(part 1 of 2)
# Autodesk Inventor assembly: 0008-10-01 Sckeleton
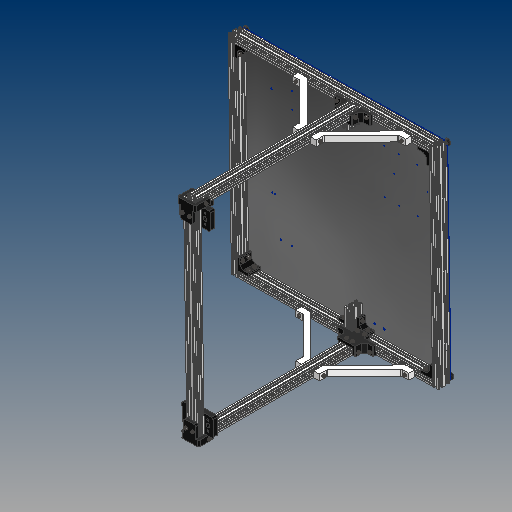
[picture p0: Inventor's stored thumbnail of the model, 512x512]
Saved by Autodesk Inventor 2020.2 (Build 242310000, 310)
## iProperties
Created: 2021-02-20
Part Number: 0008-10-01 Sckeleton
Document SubType Name: Assembly
Designer: Iulian Bors
Description: Scheleton
Author: Iulian Bors
Subject: 10-01
## Documents named in this file (20)
- Z:\I.A.B\Proiecte\0008 I.A.B 3D 2.1 Imprimanta aracet Metal\10 Mecanic\0008-10-01 Sckeleton.iam
- Z:\I.A.B\Proiecte\0008 I.A.B 3D 2.1 Imprimanta aracet Metal\10 Mecanic\0008-10-1018 V slot profiles.ipt
- Z:\I.A.B\Proiecte\0008 I.A.B 3D 2.1 Imprimanta aracet Metal\10 Mecanic\0008-10-1019 V slot profiles.ipt
- Z:\I.A.B\Proiecte\0008 I.A.B 3D 2.1 Imprimanta aracet Metal\10 Mecanic\0008-10-1020 V slot profiles.ipt
- Z:\I.A.B\Proiecte\0008 I.A.B 3D 2.1 Imprimanta aracet Metal\10 Mecanic\0008-10-1021  V slot profiles.ipt
- Z:\I.A.B\Proiecte\0008 I.A.B 3D 2.1 Imprimanta aracet Metal\10 Mecanic\0008-10-022 Tabla suport.ipt
- Z:\I.A.B\Proiecte\0008 I.A.B 3D 2.1 Imprimanta aracet Metal\10 Mecanic\0008-10-023 Suport L.ipt
- Z:\I.A.B\Proiecte\0008 I.A.B 3D 2.1 Imprimanta aracet Metal\10 Mecanic\0008-10-024 Ranforsare.ipt
- Z:\I.A.B\Proiecte\0008 I.A.B 3D 2.1 Imprimanta aracet Metal\10 Mecanic\0008-10-030 Suport L.ipt
- Z:\I.A.B\Proiecte\0008 I.A.B 3D 2.1 Imprimanta aracet Metal\10 Mecanic\0008-10-031 Suport L + placa.ipt
- Z:\I.A.B\Proiecte\0008 I.A.B 3D 2.1 Imprimanta aracet Metal\10 Mecanic\0008-10-032 Suport cadru si axa Z.ipt
- Z:\I.A.B\Proiecte\0008 I.A.B 3D 2.1 Imprimanta aracet Metal\10 Mecanic\0008-10-033.ipt
- Z:\I.A.B\Proiecte\0008 I.A.B 3D 2.1 Imprimanta aracet Metal\10 Mecanic\0008-10-035.ipt
- Z:\I.A.B\Proiecte\0008 I.A.B 3D 2.1 Imprimanta aracet Metal\10 Mecanic\0008-10-053 picior.ipt
- Z:\I.A.B\Proiecte\0008 I.A.B 3D 2.1 Imprimanta aracet Metal\10 Mecanic\0008-10-2010 M 5 Canal.ipt
- Z:\I.A.B\Proiecte\0008 I.A.B 3D 2.1 Imprimanta aracet Metal\10 Mecanic\0008-10-2011 DIN 7984 - M5 x 16.ipt
- Z:\I.A.B\Proiecte\0008 I.A.B 3D 2.1 Imprimanta aracet Metal\10 Mecanic\0008-10-2012 DIN 125 - A 5.3.ipt
- Z:\I.A.B\Proiecte\0008 I.A.B 3D 2.1 Imprimanta aracet Metal\10 Mecanic\0008-10-2013 DIN 7984 - M5 x 20.ipt
- Z:\I.A.B\Proiecte\0008 I.A.B 3D 2.1 Imprimanta aracet Metal\10 Mecanic\0008-10-2014 DIN 7984 - M5 x 25.ipt
- Z:\I.A.B\Proiecte\0008 I.A.B 3D 2.1 Imprimanta aracet Metal\10 Mecanic\0008-10-2015 DIN 7984 - M5 x 8.ipt
## Components (272 placed, 19 different names)
1. 0008-10-1018 V slot profiles.ipt:1 — Flush:78, Mate:85, Flush:79, Flush:80, Mate:86, Flush:81, Mate:109, Flush:101, Mate:112, Mate:114
2. 0008-10-1019 V slot profiles.ipt:2 — Flush:78, Mate:85, Flush:79, Mate:100, Flush:96, Mate:105, Flush:102, Mate:111, Flush:104, Mate:122, Mate:123, Flush:105, Mate:125, Flush:106, Mate:152, Mate:156, Mate:157
3. 0008-10-1019 V slot profiles.ipt:3 — Flush:80, Mate:86, Flush:81, Flush:82, Flush:85, Mate:90, Mate:99, Flush:95, Mate:106, Flush:100, Mate:116, Mate:119, Mate:127, Mate:132, Mate:143, Flush:114, Mate:146, Mate:149
4. 0008-10-1018 V slot profiles.ipt:4 — Flush:82, Flush:85, Mate:90, Flush:103, Mate:118, Mate:121
5. 0008-10-1018 V slot profiles.ipt:5 — Flush:97, Flush:98, Mate:110, Mate:161, Mate:165, Flush:116, Mate:170, Mate:177
6. 0008-10-1020 V slot profiles.ipt:6 — Flush:91, Mate:99, Flush:95, Flush:97, Flush:98, Mate:128, Flush:107, Mate:131, Flush:109, Mate:144, Mate:169, Flush:117, Flush:118, Mate:178
7. 0008-10-1020 V slot profiles.ipt:7 — Flush:91, Mate:100, Flush:96, Flush:103, Mate:110, Mate:124, Mate:126, Mate:158, Mate:159, Mate:162, Flush:115, Mate:166
8. 0008-10-1021  V slot profiles.ipt:8 — Mate:105, Mate:153, Mate:155, Flush:132
9. 0008-10-1021  V slot profiles.ipt:9 — Mate:106, Flush:100, Mate:147, Mate:150, Flush:132
10. 0008-10-022 Tabla suport.ipt:10 — Mate:109, Flush:101, Flush:102, Mate:115, Mate:117, Mate:120, Mate:145, Mate:148, Mate:151, Mate:154, Insert:21, Mate:179, Mate:180, Mate:181, Insert:242, Insert:265, Insert:266, Insert:267, Insert:268, Insert:269, Insert:270, Insert:271, Insert:272, Insert:273, Insert:274, Insert:275
11. 0008-10-023 Suport L.ipt:11 — Mate:111, Flush:104, Mate:112, Insert:24, Insert:33, Insert:34, Insert:35
12. 0008-10-023 Suport L.ipt:12 — Mate:120, Mate:121, Mate:122, Insert:66, Insert:67, Insert:68, Insert:69
13. 0008-10-023 Suport L.ipt:13 — Mate:117, Mate:118, Mate:119, Insert:54, Insert:55, Insert:56, Insert:57
14. 0008-10-023 Suport L.ipt:14 — Mate:114, Mate:115, Mate:116, Insert:36, Insert:43, Insert:44, Insert:45
15. 0008-10-024 Ranforsare.ipt:15 — Mate:123, Flush:105, Mate:124, Insert:235, Insert:236
16. 0008-10-024 Ranforsare.ipt:16 — Mate:127, Mate:128, Flush:107, Insert:224, Insert:227
17. 0008-10-024 Ranforsare.ipt:17 — Mate:125, Mate:126, Flush:106, Insert:237, Insert:239
18. 0008-10-024 Ranforsare.ipt:18 — Mate:131, Flush:109, Mate:132, Insert:230, Insert:231
19. 0008-10-031 Suport L + placa.ipt:19 — Mate:143, Mate:144, Flush:114, Insert:144, Insert:145, Insert:146, Insert:147, Insert:148, Insert:149, Insert:150, Insert:153
20. 0008-10-030 Suport L.ipt:20 — Mate:145, Mate:146, Mate:147, Insert:142, Insert:143
21. 0008-10-030 Suport L.ipt:21 — Mate:148, Mate:149, Mate:150, Insert:151, Insert:152
22. 0008-10-031 Suport L + placa.ipt:22 — Mate:157, Mate:158, Mate:159, Insert:96, Insert:97, Insert:98, Insert:99, Insert:100, Insert:101, Insert:102, Insert:103
23. 0008-10-030 Suport L.ipt:23 — Mate:151, Mate:152, Mate:153, Insert:94, Insert:95
24. 0008-10-030 Suport L.ipt:24 — Mate:154, Mate:155, Mate:156, Insert:104, Insert:105
25. 0008-10-032 Suport cadru si axa Z.ipt:25 — Mate:161, Mate:162, Flush:115, Insert:174, Insert:175, Insert:176, Insert:177
26. 0008-10-033.ipt:26 — Mate:165, Flush:116, Mate:166, Insert:197, Insert:198, Insert:199, Insert:200
27. 0008-10-035.ipt:27 — Mate:169, Flush:117, Mate:170, Insert:180, Mate:182, Insert:187, Insert:188
28. 0008-10-032 Suport cadru si axa Z.ipt:28 — Mate:177, Flush:118, Mate:178, Insert:162, Insert:163, Insert:164, Insert:165
29. 0008-10-053 picior.ipt:29 — Insert:21, Insert:115
30. 0008-10-053 picior.ipt:30 — Mate:181, Insert:116
31. 0008-10-053 picior.ipt:31 — Mate:179, Insert:117
32. 0008-10-053 picior.ipt:32 — Mate:180, Insert:114
33. 0008-10-2010 M 5 Canal.ipt:33 — Insert:22
34. 0008-10-2011 DIN 7984 - M5 x 16.ipt:34 — Insert:22, Insert:23
35. 0008-10-2012 DIN 125 - A 5.3.ipt:35 — Insert:23, Insert:24
36. 0008-10-2010 M 5 Canal.ipt:36
37. 0008-10-2011 DIN 7984 - M5 x 16.ipt:37
38. 0008-10-2012 DIN 125 - A 5.3.ipt:38 — Insert:33
39. 0008-10-2010 M 5 Canal.ipt:39
40. 0008-10-2011 DIN 7984 - M5 x 16.ipt:40
41. 0008-10-2012 DIN 125 - A 5.3.ipt:41 — Insert:34
42. 0008-10-2010 M 5 Canal.ipt:42
43. 0008-10-2011 DIN 7984 - M5 x 16.ipt:43
44. 0008-10-2012 DIN 125 - A 5.3.ipt:44 — Insert:35
45. 0008-10-2010 M 5 Canal.ipt:45
46. 0008-10-2011 DIN 7984 - M5 x 16.ipt:46
47. 0008-10-2012 DIN 125 - A 5.3.ipt:47 — Insert:36
48. 0008-10-2010 M 5 Canal.ipt:48
49. 0008-10-2011 DIN 7984 - M5 x 16.ipt:49
50. 0008-10-2012 DIN 125 - A 5.3.ipt:50 — Insert:44
51. 0008-10-2010 M 5 Canal.ipt:51
52. 0008-10-2011 DIN 7984 - M5 x 16.ipt:52
53. 0008-10-2012 DIN 125 - A 5.3.ipt:53 — Insert:45
54. 0008-10-2010 M 5 Canal.ipt:54
55. 0008-10-2011 DIN 7984 - M5 x 16.ipt:55
56. 0008-10-2012 DIN 125 - A 5.3.ipt:56 — Insert:43
57. 0008-10-2010 M 5 Canal.ipt:57
58. 0008-10-2011 DIN 7984 - M5 x 16.ipt:58
59. 0008-10-2012 DIN 125 - A 5.3.ipt:59 — Insert:57
60. 0008-10-2010 M 5 Canal.ipt:60
61. 0008-10-2011 DIN 7984 - M5 x 16.ipt:61
62. 0008-10-2012 DIN 125 - A 5.3.ipt:62 — Insert:56
63. 0008-10-2010 M 5 Canal.ipt:63
64. 0008-10-2011 DIN 7984 - M5 x 16.ipt:64
65. 0008-10-2012 DIN 125 - A 5.3.ipt:65 — Insert:55
66. 0008-10-2010 M 5 Canal.ipt:66
67. 0008-10-2011 DIN 7984 - M5 x 16.ipt:67
68. 0008-10-2012 DIN 125 - A 5.3.ipt:68 — Insert:54
69. 0008-10-2010 M 5 Canal.ipt:69
70. 0008-10-2011 DIN 7984 - M5 x 16.ipt:70
71. 0008-10-2012 DIN 125 - A 5.3.ipt:71 — Insert:66
72. 0008-10-2010 M 5 Canal.ipt:72
73. 0008-10-2011 DIN 7984 - M5 x 16.ipt:73
74. 0008-10-2012 DIN 125 - A 5.3.ipt:74 — Insert:67
75. 0008-10-2010 M 5 Canal.ipt:75
76. 0008-10-2011 DIN 7984 - M5 x 16.ipt:76
77. 0008-10-2012 DIN 125 - A 5.3.ipt:77 — Insert:68
78. 0008-10-2010 M 5 Canal.ipt:78
79. 0008-10-2011 DIN 7984 - M5 x 16.ipt:79
80. 0008-10-2012 DIN 125 - A 5.3.ipt:80 — Insert:69
81. 0008-10-2010 M 5 Canal.ipt:81
82. 0008-10-2011 DIN 7984 - M5 x 16.ipt:82
83. 0008-10-2012 DIN 125 - A 5.3.ipt:83 — Insert:94
84. 0008-10-2010 M 5 Canal.ipt:84
85. 0008-10-2011 DIN 7984 - M5 x 16.ipt:85
86. 0008-10-2012 DIN 125 - A 5.3.ipt:86 — Insert:96
87. 0008-10-2010 M 5 Canal.ipt:87
88. 0008-10-2011 DIN 7984 - M5 x 16.ipt:88
89. 0008-10-2012 DIN 125 - A 5.3.ipt:89 — Insert:95
90. 0008-10-2010 M 5 Canal.ipt:90
91. 0008-10-2011 DIN 7984 - M5 x 16.ipt:91
92. 0008-10-2012 DIN 125 - A 5.3.ipt:92 — Insert:97
93. 0008-10-2010 M 5 Canal.ipt:93
94. 0008-10-2011 DIN 7984 - M5 x 16.ipt:94
95. 0008-10-2012 DIN 125 - A 5.3.ipt:95 — Insert:98
96. 0008-10-2010 M 5 Canal.ipt:96
97. 0008-10-2011 DIN 7984 - M5 x 16.ipt:97
98. 0008-10-2012 DIN 125 - A 5.3.ipt:98 — Insert:102
99. 0008-10-2010 M 5 Canal.ipt:99
100. 0008-10-2011 DIN 7984 - M5 x 16.ipt:100
101. 0008-10-2012 DIN 125 - A 5.3.ipt:101 — Insert:100
102. 0008-10-2010 M 5 Canal.ipt:102
103. 0008-10-2011 DIN 7984 - M5 x 16.ipt:103
104. 0008-10-2012 DIN 125 - A 5.3.ipt:104 — Insert:101
105. 0008-10-2010 M 5 Canal.ipt:105
106. 0008-10-2011 DIN 7984 - M5 x 16.ipt:106
107. 0008-10-2012 DIN 125 - A 5.3.ipt:107 — Insert:105
108. 0008-10-2010 M 5 Canal.ipt:108
109. 0008-10-2011 DIN 7984 - M5 x 16.ipt:109
110. 0008-10-2012 DIN 125 - A 5.3.ipt:110 — Insert:104
111. 0008-10-2010 M 5 Canal.ipt:111
112. 0008-10-2011 DIN 7984 - M5 x 16.ipt:112
113. 0008-10-2012 DIN 125 - A 5.3.ipt:113 — Insert:103
114. 0008-10-2010 M 5 Canal.ipt:114
115. 0008-10-2011 DIN 7984 - M5 x 16.ipt:115
116. 0008-10-2012 DIN 125 - A 5.3.ipt:116 — Insert:99
117. 0008-10-2010 M 5 Canal.ipt:117
118. 0008-10-2011 DIN 7984 - M5 x 16.ipt:118
119. 0008-10-2012 DIN 125 - A 5.3.ipt:119 — Insert:114
120. 0008-10-2010 M 5 Canal.ipt:120
121. 0008-10-2011 DIN 7984 - M5 x 16.ipt:121
122. 0008-10-2012 DIN 125 - A 5.3.ipt:122 — Insert:115
123. 0008-10-2010 M 5 Canal.ipt:123
124. 0008-10-2011 DIN 7984 - M5 x 16.ipt:124
125. 0008-10-2012 DIN 125 - A 5.3.ipt:125 — Insert:116
126. 0008-10-2010 M 5 Canal.ipt:126
127. 0008-10-2011 DIN 7984 - M5 x 16.ipt:127
128. 0008-10-2012 DIN 125 - A 5.3.ipt:128 — Insert:117
129. 0008-10-2010 M 5 Canal.ipt:129
130. 0008-10-2011 DIN 7984 - M5 x 16.ipt:130
131. 0008-10-2012 DIN 125 - A 5.3.ipt:131 — Insert:145
132. 0008-10-2010 M 5 Canal.ipt:132
133. 0008-10-2011 DIN 7984 - M5 x 16.ipt:133
134. 0008-10-2012 DIN 125 - A 5.3.ipt:134 — Insert:144
135. 0008-10-2010 M 5 Canal.ipt:135
136. 0008-10-2011 DIN 7984 - M5 x 16.ipt:136
137. 0008-10-2012 DIN 125 - A 5.3.ipt:137 — Insert:143
138. 0008-10-2010 M 5 Canal.ipt:138
139. 0008-10-2011 DIN 7984 - M5 x 16.ipt:139
140. 0008-10-2012 DIN 125 - A 5.3.ipt:140 — Insert:146
141. 0008-10-2010 M 5 Canal.ipt:141
142. 0008-10-2011 DIN 7984 - M5 x 16.ipt:142
143. 0008-10-2012 DIN 125 - A 5.3.ipt:143 — Insert:150
144. 0008-10-2010 M 5 Canal.ipt:144
145. 0008-10-2011 DIN 7984 - M5 x 16.ipt:145
146. 0008-10-2012 DIN 125 - A 5.3.ipt:146 — Insert:147
147. 0008-10-2010 M 5 Canal.ipt:147
148. 0008-10-2011 DIN 7984 - M5 x 16.ipt:148
149. 0008-10-2012 DIN 125 - A 5.3.ipt:149 — Insert:153
150. 0008-10-2010 M 5 Canal.ipt:150
151. 0008-10-2011 DIN 7984 - M5 x 16.ipt:151
152. 0008-10-2012 DIN 125 - A 5.3.ipt:152 — Insert:152
153. 0008-10-2010 M 5 Canal.ipt:153
154. 0008-10-2011 DIN 7984 - M5 x 16.ipt:154
155. 0008-10-2012 DIN 125 - A 5.3.ipt:155 — Insert:151
156. 0008-10-2010 M 5 Canal.ipt:156
157. 0008-10-2011 DIN 7984 - M5 x 16.ipt:157
158. 0008-10-2012 DIN 125 - A 5.3.ipt:158 — Insert:149
159. 0008-10-2010 M 5 Canal.ipt:159
160. 0008-10-2011 DIN 7984 - M5 x 16.ipt:160
161. 0008-10-2012 DIN 125 - A 5.3.ipt:161 — Insert:148
162. 0008-10-2010 M 5 Canal.ipt:162
163. 0008-10-2011 DIN 7984 - M5 x 16.ipt:163
164. 0008-10-2012 DIN 125 - A 5.3.ipt:164 — Insert:142
165. 0008-10-2010 M 5 Canal.ipt:165
166. 0008-10-2011 DIN 7984 - M5 x 16.ipt:166
167. 0008-10-2012 DIN 125 - A 5.3.ipt:167 — Insert:162
168. 0008-10-2010 M 5 Canal.ipt:168
169. 0008-10-2011 DIN 7984 - M5 x 16.ipt:169
170. 0008-10-2012 DIN 125 - A 5.3.ipt:170 — Insert:163
171. 0008-10-2010 M 5 Canal.ipt:171
172. 0008-10-2011 DIN 7984 - M5 x 16.ipt:172
173. 0008-10-2012 DIN 125 - A 5.3.ipt:173 — Insert:165
174. 0008-10-2010 M 5 Canal.ipt:174
175. 0008-10-2011 DIN 7984 - M5 x 16.ipt:175
176. 0008-10-2012 DIN 125 - A 5.3.ipt:176 — Insert:164
177. 0008-10-2010 M 5 Canal.ipt:177
178. 0008-10-2011 DIN 7984 - M5 x 16.ipt:178
179. 0008-10-2012 DIN 125 - A 5.3.ipt:179 — Insert:174
180. 0008-10-2010 M 5 Canal.ipt:180
181. 0008-10-2011 DIN 7984 - M5 x 16.ipt:181
182. 0008-10-2012 DIN 125 - A 5.3.ipt:182 — Insert:176
183. 0008-10-2010 M 5 Canal.ipt:183
184. 0008-10-2011 DIN 7984 - M5 x 16.ipt:184
185. 0008-10-2012 DIN 125 - A 5.3.ipt:185 — Insert:175
186. 0008-10-2010 M 5 Canal.ipt:186
187. 0008-10-2011 DIN 7984 - M5 x 16.ipt:187
188. 0008-10-2012 DIN 125 - A 5.3.ipt:188 — Insert:177
189. 0008-10-2010 M 5 Canal.ipt:189 — Insert:178
190. 0008-10-2012 DIN 125 - A 5.3.ipt:190 — Insert:179, Insert:180
191. 0008-10-2013 DIN 7984 - M5 x 20.ipt:191 — Insert:178, Insert:179
192. 0008-10-2010 M 5 Canal.ipt:192
193. 0008-10-2012 DIN 125 - A 5.3.ipt:193 — Mate:182
194. 0008-10-2013 DIN 7984 - M5 x 20.ipt:194
195. 0008-10-2010 M 5 Canal.ipt:195
196. 0008-10-2012 DIN 125 - A 5.3.ipt:196 — Insert:188
197. 0008-10-2013 DIN 7984 - M5 x 20.ipt:197
198. 0008-10-2010 M 5 Canal.ipt:198
199. 0008-10-2012 DIN 125 - A 5.3.ipt:199 — Insert:187
200. 0008-10-2013 DIN 7984 - M5 x 20.ipt:200
201. 0008-10-2010 M 5 Canal.ipt:201
202. 0008-10-2012 DIN 125 - A 5.3.ipt:202 — Insert:198
203. 0008-10-2013 DIN 7984 - M5 x 20.ipt:203
204. 0008-10-2010 M 5 Canal.ipt:204
205. 0008-10-2012 DIN 125 - A 5.3.ipt:205 — Insert:200
206. 0008-10-2013 DIN 7984 - M5 x 20.ipt:206
207. 0008-10-2010 M 5 Canal.ipt:207
208. 0008-10-2012 DIN 125 - A 5.3.ipt:208 — Insert:199
209. 0008-10-2013 DIN 7984 - M5 x 20.ipt:209
210. 0008-10-2010 M 5 Canal.ipt:210
211. 0008-10-2012 DIN 125 - A 5.3.ipt:211 — Insert:197
212. 0008-10-2013 DIN 7984 - M5 x 20.ipt:212
213. 0008-10-2010 M 5 Canal.ipt:213
214. 0008-10-2010 M 5 Canal.ipt:214
215. 0008-10-2010 M 5 Canal.ipt:215
216. 0008-10-2010 M 5 Canal.ipt:216
217. 0008-10-2010 M 5 Canal.ipt:217
218. 0008-10-2012 DIN 125 - A 5.3.ipt:218 — Insert:224, Insert:225
219. 0008-10-2010 M 5 Canal.ipt:219
220. 0008-10-2010 M 5 Canal.ipt:220
221. 0008-10-2010 M 5 Canal.ipt:221
222. 0008-10-2014 DIN 7984 - M5 x 25.ipt:222 — Insert:225
223. 0008-10-2012 DIN 125 - A 5.3.ipt:223 — Insert:227
224. 0008-10-2014 DIN 7984 - M5 x 25.ipt:224
225. 0008-10-2012 DIN 125 - A 5.3.ipt:225 — Insert:231
226. 0008-10-2014 DIN 7984 - M5 x 25.ipt:226
227. 0008-10-2012 DIN 125 - A 5.3.ipt:227 — Insert:230
228. 0008-10-2014 DIN 7984 - M5 x 25.ipt:228
229. 0008-10-2012 DIN 125 - A 5.3.ipt:229 — Insert:237
230. 0008-10-2014 DIN 7984 - M5 x 25.ipt:230
231. 0008-10-2012 DIN 125 - A 5.3.ipt:231 — Insert:236
232. 0008-10-2014 DIN 7984 - M5 x 25.ipt:232
233. 0008-10-2012 DIN 125 - A 5.3.ipt:233 — Insert:235
234. 0008-10-2014 DIN 7984 - M5 x 25.ipt:234
235. 0008-10-2012 DIN 125 - A 5.3.ipt:235 — Insert:239
236. 0008-10-2014 DIN 7984 - M5 x 25.ipt:236
237. 0008-10-2010 M 5 Canal.ipt:237 — Insert:240
238. 0008-10-2012 DIN 125 - A 5.3.ipt:238 — Insert:241, Insert:242
239. 0008-10-2015 DIN 7984 - M5 x 8.ipt:239 — Insert:240, Insert:241
240. 0008-10-2010 M 5 Canal.ipt:240
241. 0008-10-2012 DIN 125 - A 5.3.ipt:241 — Insert:265
242. 0008-10-2015 DIN 7984 - M5 x 8.ipt:242
243. 0008-10-2010 M 5 Canal.ipt:243
244. 0008-10-2012 DIN 125 - A 5.3.ipt:244 — Insert:266
245. 0008-10-2015 DIN 7984 - M5 x 8.ipt:245
246. 0008-10-2010 M 5 Canal.ipt:246
247. 0008-10-2012 DIN 125 - A 5.3.ipt:247 — Insert:267
248. 0008-10-2015 DIN 7984 - M5 x 8.ipt:248
249. 0008-10-2010 M 5 Canal.ipt:249
250. 0008-10-2012 DIN 125 - A 5.3.ipt:250 — Insert:268
251. 0008-10-2015 DIN 7984 - M5 x 8.ipt:251
252. 0008-10-2010 M 5 Canal.ipt:252
253. 0008-10-2012 DIN 125 - A 5.3.ipt:253 — Insert:269
254. 0008-10-2015 DIN 7984 - M5 x 8.ipt:254
255. 0008-10-2010 M 5 Canal.ipt:255
256. 0008-10-2012 DIN 125 - A 5.3.ipt:256 — Insert:270
257. 0008-10-2015 DIN 7984 - M5 x 8.ipt:257
258. 0008-10-2010 M 5 Canal.ipt:258
259. 0008-10-2012 DIN 125 - A 5.3.ipt:259 — Insert:272
260. 0008-10-2015 DIN 7984 - M5 x 8.ipt:260
261. 0008-10-2010 M 5 Canal.ipt:261
262. 0008-10-2012 DIN 125 - A 5.3.ipt:262 — Insert:273
263. 0008-10-2015 DIN 7984 - M5 x 8.ipt:263
264. 0008-10-2010 M 5 Canal.ipt:264
265. 0008-10-2012 DIN 125 - A 5.3.ipt:265 — Insert:274
266. 0008-10-2015 DIN 7984 - M5 x 8.ipt:266
267. 0008-10-2010 M 5 Canal.ipt:267
268. 0008-10-2012 DIN 125 - A 5.3.ipt:268 — Insert:271
269. 0008-10-2015 DIN 7984 - M5 x 8.ipt:269
270. 0008-10-2010 M 5 Canal.ipt:270
271. 0008-10-2012 DIN 125 - A 5.3.ipt:271 — Insert:275
272. 0008-10-2015 DIN 7984 - M5 x 8.ipt:272
## Relationships (315: Insert 232, Mate 57, Flush 26)
- Flush:78: 0008-10-1018 V slot profiles.ipt:1 ↔ 0008-10-1019 V slot profiles.ipt:2
- Mate:85: 0008-10-1018 V slot profiles.ipt:1 ↔ 0008-10-1019 V slot profiles.ipt:2
- Flush:79: 0008-10-1018 V slot profiles.ipt:1 ↔ 0008-10-1019 V slot profiles.ipt:2
- Flush:80: 0008-10-1018 V slot profiles.ipt:1 ↔ 0008-10-1019 V slot profiles.ipt:3
- Mate:86: 0008-10-1018 V slot profiles.ipt:1 ↔ 0008-10-1019 V slot profiles.ipt:3
- Flush:81: 0008-10-1018 V slot profiles.ipt:1 ↔ 0008-10-1019 V slot profiles.ipt:3
- Flush:82: 0008-10-1019 V slot profiles.ipt:3 ↔ 0008-10-1018 V slot profiles.ipt:4
- Flush:85: 0008-10-1019 V slot profiles.ipt:3 ↔ 0008-10-1018 V slot profiles.ipt:4
- Mate:90: 0008-10-1019 V slot profiles.ipt:3 ↔ 0008-10-1018 V slot profiles.ipt:4
- Flush:91: 0008-10-1020 V slot profiles.ipt:6 ↔ 0008-10-1020 V slot profiles.ipt:7
- Mate:99: 0008-10-1019 V slot profiles.ipt:3 ↔ 0008-10-1020 V slot profiles.ipt:6
- Flush:95: 0008-10-1019 V slot profiles.ipt:3 ↔ 0008-10-1020 V slot profiles.ipt:6
- Mate:100: 0008-10-1019 V slot profiles.ipt:2 ↔ 0008-10-1020 V slot profiles.ipt:7
- Flush:96: 0008-10-1019 V slot profiles.ipt:2 ↔ 0008-10-1020 V slot profiles.ipt:7
- Flush:97: 0008-10-1018 V slot profiles.ipt:5 ↔ 0008-10-1020 V slot profiles.ipt:6
- Flush:98: 0008-10-1018 V slot profiles.ipt:5 ↔ 0008-10-1020 V slot profiles.ipt:6
- Mate:105: 0008-10-1019 V slot profiles.ipt:2 ↔ 0008-10-1021  V slot profiles.ipt:8
- Mate:106: 0008-10-1019 V slot profiles.ipt:3 ↔ 0008-10-1021  V slot profiles.ipt:9
- Flush:100: 0008-10-1019 V slot profiles.ipt:3 ↔ 0008-10-1021  V slot profiles.ipt:9
- Mate:109: 0008-10-1018 V slot profiles.ipt:1 ↔ 0008-10-022 Tabla suport.ipt:10
- Flush:101: 0008-10-1018 V slot profiles.ipt:1 ↔ 0008-10-022 Tabla suport.ipt:10
- Flush:102: 0008-10-1019 V slot profiles.ipt:2 ↔ 0008-10-022 Tabla suport.ipt:10
- Flush:103 (250.528 mm): 0008-10-1018 V slot profiles.ipt:4 ↔ 0008-10-1020 V slot profiles.ipt:7
- Mate:110: 0008-10-1018 V slot profiles.ipt:5 ↔ 0008-10-1020 V slot profiles.ipt:7
- Mate:111: 0008-10-1019 V slot profiles.ipt:2 ↔ 0008-10-023 Suport L.ipt:11
- Flush:104: 0008-10-1019 V slot profiles.ipt:2 ↔ 0008-10-023 Suport L.ipt:11
- Mate:112: 0008-10-1018 V slot profiles.ipt:1 ↔ 0008-10-023 Suport L.ipt:11
- Mate:114: 0008-10-1018 V slot profiles.ipt:1 ↔ 0008-10-023 Suport L.ipt:14
- Mate:115: 0008-10-022 Tabla suport.ipt:10 ↔ 0008-10-023 Suport L.ipt:14
- Mate:116: 0008-10-1019 V slot profiles.ipt:3 ↔ 0008-10-023 Suport L.ipt:14
- Mate:117: 0008-10-022 Tabla suport.ipt:10 ↔ 0008-10-023 Suport L.ipt:13
- Mate:118: 0008-10-1018 V slot profiles.ipt:4 ↔ 0008-10-023 Suport L.ipt:13
- Mate:119: 0008-10-1019 V slot profiles.ipt:3 ↔ 0008-10-023 Suport L.ipt:13
- Mate:120: 0008-10-022 Tabla suport.ipt:10 ↔ 0008-10-023 Suport L.ipt:12
- Mate:121: 0008-10-1018 V slot profiles.ipt:4 ↔ 0008-10-023 Suport L.ipt:12
- Mate:122: 0008-10-1019 V slot profiles.ipt:2 ↔ 0008-10-023 Suport L.ipt:12
- Mate:123: 0008-10-1019 V slot profiles.ipt:2 ↔ 0008-10-024 Ranforsare.ipt:15
- Flush:105: 0008-10-1019 V slot profiles.ipt:2 ↔ 0008-10-024 Ranforsare.ipt:15
- Mate:124: 0008-10-1020 V slot profiles.ipt:7 ↔ 0008-10-024 Ranforsare.ipt:15
- Mate:125: 0008-10-1019 V slot profiles.ipt:2 ↔ 0008-10-024 Ranforsare.ipt:17
- Mate:126: 0008-10-1020 V slot profiles.ipt:7 ↔ 0008-10-024 Ranforsare.ipt:17
- Flush:106: 0008-10-1019 V slot profiles.ipt:2 ↔ 0008-10-024 Ranforsare.ipt:17
- Mate:127: 0008-10-1019 V slot profiles.ipt:3 ↔ 0008-10-024 Ranforsare.ipt:16
- Mate:128: 0008-10-1020 V slot profiles.ipt:6 ↔ 0008-10-024 Ranforsare.ipt:16
- Flush:107: 0008-10-1020 V slot profiles.ipt:6 ↔ 0008-10-024 Ranforsare.ipt:16
- Mate:131: 0008-10-1020 V slot profiles.ipt:6 ↔ 0008-10-024 Ranforsare.ipt:18
- Flush:109: 0008-10-1020 V slot profiles.ipt:6 ↔ 0008-10-024 Ranforsare.ipt:18
- Mate:132: 0008-10-1019 V slot profiles.ipt:3 ↔ 0008-10-024 Ranforsare.ipt:18
- Mate:143: 0008-10-1019 V slot profiles.ipt:3 ↔ 0008-10-031 Suport L + placa.ipt:19
- Mate:144: 0008-10-1020 V slot profiles.ipt:6 ↔ 0008-10-031 Suport L + placa.ipt:19
- Flush:114: 0008-10-1019 V slot profiles.ipt:3 ↔ 0008-10-031 Suport L + placa.ipt:19
- Mate:145: 0008-10-022 Tabla suport.ipt:10 ↔ 0008-10-030 Suport L.ipt:20
- Mate:146: 0008-10-1019 V slot profiles.ipt:3 ↔ 0008-10-030 Suport L.ipt:20
- Mate:147: 0008-10-1021  V slot profiles.ipt:9 ↔ 0008-10-030 Suport L.ipt:20
- Mate:148: 0008-10-022 Tabla suport.ipt:10 ↔ 0008-10-030 Suport L.ipt:21
- Mate:149: 0008-10-1019 V slot profiles.ipt:3 ↔ 0008-10-030 Suport L.ipt:21
- Mate:150: 0008-10-1021  V slot profiles.ipt:9 ↔ 0008-10-030 Suport L.ipt:21
- Mate:151: 0008-10-022 Tabla suport.ipt:10 ↔ 0008-10-030 Suport L.ipt:23
- Mate:152: 0008-10-1019 V slot profiles.ipt:2 ↔ 0008-10-030 Suport L.ipt:23
- Mate:153: 0008-10-1021  V slot profiles.ipt:8 ↔ 0008-10-030 Suport L.ipt:23
- Mate:154: 0008-10-022 Tabla suport.ipt:10 ↔ 0008-10-030 Suport L.ipt:24
- Mate:155: 0008-10-1021  V slot profiles.ipt:8 ↔ 0008-10-030 Suport L.ipt:24
- Mate:156: 0008-10-1019 V slot profiles.ipt:2 ↔ 0008-10-030 Suport L.ipt:24
- Mate:157: 0008-10-1019 V slot profiles.ipt:2 ↔ 0008-10-031 Suport L + placa.ipt:22
- Mate:158: 0008-10-1020 V slot profiles.ipt:7 ↔ 0008-10-031 Suport L + placa.ipt:22
- Mate:159: 0008-10-1020 V slot profiles.ipt:7 ↔ 0008-10-031 Suport L + placa.ipt:22
- Mate:161: 0008-10-1018 V slot profiles.ipt:5 ↔ 0008-10-032 Suport cadru si axa Z.ipt:25
- Mate:162 (0.15 mm): 0008-10-1020 V slot profiles.ipt:7 ↔ 0008-10-032 Suport cadru si axa Z.ipt:25
- Flush:115: 0008-10-1020 V slot profiles.ipt:7 ↔ 0008-10-032 Suport cadru si axa Z.ipt:25
- Mate:165: 0008-10-1018 V slot profiles.ipt:5 ↔ 0008-10-033.ipt:26
- Flush:116: 0008-10-1018 V slot profiles.ipt:5 ↔ 0008-10-033.ipt:26
- Mate:166: 0008-10-1020 V slot profiles.ipt:7 ↔ 0008-10-033.ipt:26
- Mate:169: 0008-10-1020 V slot profiles.ipt:6 ↔ 0008-10-035.ipt:27
- Flush:117: 0008-10-1020 V slot profiles.ipt:6 ↔ 0008-10-035.ipt:27
- Mate:170: 0008-10-1018 V slot profiles.ipt:5 ↔ 0008-10-035.ipt:27
- Mate:177: 0008-10-1018 V slot profiles.ipt:5 ↔ 0008-10-032 Suport cadru si axa Z.ipt:28
- Flush:118: 0008-10-1020 V slot profiles.ipt:6 ↔ 0008-10-032 Suport cadru si axa Z.ipt:28
- Mate:178: 0008-10-1020 V slot profiles.ipt:6 ↔ 0008-10-032 Suport cadru si axa Z.ipt:28
- Flush:132: 0008-10-1021  V slot profiles.ipt:8 ↔ 0008-10-1021  V slot profiles.ipt:9
- Insert:21: 0008-10-022 Tabla suport.ipt:10 ↔ 0008-10-053 picior.ipt:29
- Mate:179: 0008-10-022 Tabla suport.ipt:10 ↔ 0008-10-053 picior.ipt:31
- Mate:180: 0008-10-022 Tabla suport.ipt:10 ↔ 0008-10-053 picior.ipt:32
- Mate:181: 0008-10-022 Tabla suport.ipt:10 ↔ 0008-10-053 picior.ipt:30
- Insert:22 (-5 mm): 0008-10-2010 M 5 Canal.ipt:33 ↔ 0008-10-2011 DIN 7984 - M5 x 16.ipt:34
- Insert:23: 0008-10-2011 DIN 7984 - M5 x 16.ipt:34 ↔ 0008-10-2012 DIN 125 - A 5.3.ipt:35
- Insert:24: 0008-10-023 Suport L.ipt:11 ↔ 0008-10-2012 DIN 125 - A 5.3.ipt:35
- [Insert] (-5 mm): 0008-10-2010 M 5 Canal.ipt:36 ↔ 0008-10-2011 DIN 7984 - M5 x 16.ipt:37
- [Insert]: 0008-10-2011 DIN 7984 - M5 x 16.ipt:37 ↔ 0008-10-2012 DIN 125 - A 5.3.ipt:38
- [Insert] (-5 mm): 0008-10-2010 M 5 Canal.ipt:39 ↔ 0008-10-2011 DIN 7984 - M5 x 16.ipt:40
- [Insert]: 0008-10-2011 DIN 7984 - M5 x 16.ipt:40 ↔ 0008-10-2012 DIN 125 - A 5.3.ipt:41
- [Insert] (-5 mm): 0008-10-2010 M 5 Canal.ipt:42 ↔ 0008-10-2011 DIN 7984 - M5 x 16.ipt:43
- [Insert]: 0008-10-2011 DIN 7984 - M5 x 16.ipt:43 ↔ 0008-10-2012 DIN 125 - A 5.3.ipt:44
- [Insert] (-5 mm): 0008-10-2010 M 5 Canal.ipt:45 ↔ 0008-10-2011 DIN 7984 - M5 x 16.ipt:46
- [Insert]: 0008-10-2011 DIN 7984 - M5 x 16.ipt:46 ↔ 0008-10-2012 DIN 125 - A 5.3.ipt:47
- Insert:33: 0008-10-023 Suport L.ipt:11 ↔ 0008-10-2012 DIN 125 - A 5.3.ipt:38
- Insert:34: 0008-10-023 Suport L.ipt:11 ↔ 0008-10-2012 DIN 125 - A 5.3.ipt:41
- Insert:35: 0008-10-023 Suport L.ipt:11 ↔ 0008-10-2012 DIN 125 - A 5.3.ipt:44
- Insert:36: 0008-10-023 Suport L.ipt:14 ↔ 0008-10-2012 DIN 125 - A 5.3.ipt:47
- [Insert] (-5 mm): 0008-10-2010 M 5 Canal.ipt:48 ↔ 0008-10-2011 DIN 7984 - M5 x 16.ipt:49
- [Insert]: 0008-10-2011 DIN 7984 - M5 x 16.ipt:49 ↔ 0008-10-2012 DIN 125 - A 5.3.ipt:50
- [Insert] (-5 mm): 0008-10-2010 M 5 Canal.ipt:51 ↔ 0008-10-2011 DIN 7984 - M5 x 16.ipt:52
- [Insert]: 0008-10-2011 DIN 7984 - M5 x 16.ipt:52 ↔ 0008-10-2012 DIN 125 - A 5.3.ipt:53
- [Insert] (-5 mm): 0008-10-2010 M 5 Canal.ipt:54 ↔ 0008-10-2011 DIN 7984 - M5 x 16.ipt:55
- [Insert]: 0008-10-2011 DIN 7984 - M5 x 16.ipt:55 ↔ 0008-10-2012 DIN 125 - A 5.3.ipt:56
- Insert:43: 0008-10-023 Suport L.ipt:14 ↔ 0008-10-2012 DIN 125 - A 5.3.ipt:56
- Insert:44: 0008-10-023 Suport L.ipt:14 ↔ 0008-10-2012 DIN 125 - A 5.3.ipt:50
- Insert:45: 0008-10-023 Suport L.ipt:14 ↔ 0008-10-2012 DIN 125 - A 5.3.ipt:53
- [Insert] (-5 mm): 0008-10-2010 M 5 Canal.ipt:57 ↔ 0008-10-2011 DIN 7984 - M5 x 16.ipt:58
- [Insert]: 0008-10-2011 DIN 7984 - M5 x 16.ipt:58 ↔ 0008-10-2012 DIN 125 - A 5.3.ipt:59
- [Insert] (-5 mm): 0008-10-2010 M 5 Canal.ipt:60 ↔ 0008-10-2011 DIN 7984 - M5 x 16.ipt:61
- [Insert]: 0008-10-2011 DIN 7984 - M5 x 16.ipt:61 ↔ 0008-10-2012 DIN 125 - A 5.3.ipt:62
- [Insert] (-5 mm): 0008-10-2010 M 5 Canal.ipt:63 ↔ 0008-10-2011 DIN 7984 - M5 x 16.ipt:64
- [Insert]: 0008-10-2011 DIN 7984 - M5 x 16.ipt:64 ↔ 0008-10-2012 DIN 125 - A 5.3.ipt:65
- [Insert] (-5 mm): 0008-10-2010 M 5 Canal.ipt:66 ↔ 0008-10-2011 DIN 7984 - M5 x 16.ipt:67
- [Insert]: 0008-10-2011 DIN 7984 - M5 x 16.ipt:67 ↔ 0008-10-2012 DIN 125 - A 5.3.ipt:68
- Insert:54: 0008-10-023 Suport L.ipt:13 ↔ 0008-10-2012 DIN 125 - A 5.3.ipt:68
- Insert:55: 0008-10-023 Suport L.ipt:13 ↔ 0008-10-2012 DIN 125 - A 5.3.ipt:65
- Insert:56: 0008-10-023 Suport L.ipt:13 ↔ 0008-10-2012 DIN 125 - A 5.3.ipt:62
- Insert:57: 0008-10-023 Suport L.ipt:13 ↔ 0008-10-2012 DIN 125 - A 5.3.ipt:59
- [Insert] (-5 mm): 0008-10-2010 M 5 Canal.ipt:69 ↔ 0008-10-2011 DIN 7984 - M5 x 16.ipt:70
- [Insert]: 0008-10-2011 DIN 7984 - M5 x 16.ipt:70 ↔ 0008-10-2012 DIN 125 - A 5.3.ipt:71
- [Insert] (-5 mm): 0008-10-2010 M 5 Canal.ipt:72 ↔ 0008-10-2011 DIN 7984 - M5 x 16.ipt:73
- [Insert]: 0008-10-2011 DIN 7984 - M5 x 16.ipt:73 ↔ 0008-10-2012 DIN 125 - A 5.3.ipt:74
- [Insert] (-5 mm): 0008-10-2010 M 5 Canal.ipt:75 ↔ 0008-10-2011 DIN 7984 - M5 x 16.ipt:76
- [Insert]: 0008-10-2011 DIN 7984 - M5 x 16.ipt:76 ↔ 0008-10-2012 DIN 125 - A 5.3.ipt:77
- [Insert] (-5 mm): 0008-10-2010 M 5 Canal.ipt:78 ↔ 0008-10-2011 DIN 7984 - M5 x 16.ipt:79
- [Insert]: 0008-10-2011 DIN 7984 - M5 x 16.ipt:79 ↔ 0008-10-2012 DIN 125 - A 5.3.ipt:80
- Insert:66: 0008-10-023 Suport L.ipt:12 ↔ 0008-10-2012 DIN 125 - A 5.3.ipt:71
- Insert:67: 0008-10-023 Suport L.ipt:12 ↔ 0008-10-2012 DIN 125 - A 5.3.ipt:74
- Insert:68: 0008-10-023 Suport L.ipt:12 ↔ 0008-10-2012 DIN 125 - A 5.3.ipt:77
- Insert:69: 0008-10-023 Suport L.ipt:12 ↔ 0008-10-2012 DIN 125 - A 5.3.ipt:80
- [Insert] (-5 mm): 0008-10-2010 M 5 Canal.ipt:81 ↔ 0008-10-2011 DIN 7984 - M5 x 16.ipt:82
- [Insert]: 0008-10-2011 DIN 7984 - M5 x 16.ipt:82 ↔ 0008-10-2012 DIN 125 - A 5.3.ipt:83
- [Insert] (-5 mm): 0008-10-2010 M 5 Canal.ipt:84 ↔ 0008-10-2011 DIN 7984 - M5 x 16.ipt:85
- [Insert]: 0008-10-2011 DIN 7984 - M5 x 16.ipt:85 ↔ 0008-10-2012 DIN 125 - A 5.3.ipt:86
- [Insert] (-5 mm): 0008-10-2010 M 5 Canal.ipt:87 ↔ 0008-10-2011 DIN 7984 - M5 x 16.ipt:88
- [Insert]: 0008-10-2011 DIN 7984 - M5 x 16.ipt:88 ↔ 0008-10-2012 DIN 125 - A 5.3.ipt:89
- [Insert] (-5 mm): 0008-10-2010 M 5 Canal.ipt:90 ↔ 0008-10-2011 DIN 7984 - M5 x 16.ipt:91
- [Insert]: 0008-10-2011 DIN 7984 - M5 x 16.ipt:91 ↔ 0008-10-2012 DIN 125 - A 5.3.ipt:92
- [Insert] (-5 mm): 0008-10-2010 M 5 Canal.ipt:93 ↔ 0008-10-2011 DIN 7984 - M5 x 16.ipt:94
- [Insert]: 0008-10-2011 DIN 7984 - M5 x 16.ipt:94 ↔ 0008-10-2012 DIN 125 - A 5.3.ipt:95
- [Insert] (-5 mm): 0008-10-2010 M 5 Canal.ipt:96 ↔ 0008-10-2011 DIN 7984 - M5 x 16.ipt:97
- [Insert]: 0008-10-2011 DIN 7984 - M5 x 16.ipt:97 ↔ 0008-10-2012 DIN 125 - A 5.3.ipt:98
- [Insert] (-5 mm): 0008-10-2010 M 5 Canal.ipt:99 ↔ 0008-10-2011 DIN 7984 - M5 x 16.ipt:100
- [Insert]: 0008-10-2011 DIN 7984 - M5 x 16.ipt:100 ↔ 0008-10-2012 DIN 125 - A 5.3.ipt:101
- [Insert] (-5 mm): 0008-10-2010 M 5 Canal.ipt:102 ↔ 0008-10-2011 DIN 7984 - M5 x 16.ipt:103
- [Insert]: 0008-10-2011 DIN 7984 - M5 x 16.ipt:103 ↔ 0008-10-2012 DIN 125 - A 5.3.ipt:104
- [Insert] (-5 mm): 0008-10-2010 M 5 Canal.ipt:105 ↔ 0008-10-2011 DIN 7984 - M5 x 16.ipt:106
- [Insert]: 0008-10-2011 DIN 7984 - M5 x 16.ipt:106 ↔ 0008-10-2012 DIN 125 - A 5.3.ipt:107
- [Insert] (-5 mm): 0008-10-2010 M 5 Canal.ipt:108 ↔ 0008-10-2011 DIN 7984 - M5 x 16.ipt:109
- [Insert]: 0008-10-2011 DIN 7984 - M5 x 16.ipt:109 ↔ 0008-10-2012 DIN 125 - A 5.3.ipt:110
- [Insert] (-5 mm): 0008-10-2010 M 5 Canal.ipt:111 ↔ 0008-10-2011 DIN 7984 - M5 x 16.ipt:112
- [Insert]: 0008-10-2011 DIN 7984 - M5 x 16.ipt:112 ↔ 0008-10-2012 DIN 125 - A 5.3.ipt:113
- [Insert] (-5 mm): 0008-10-2010 M 5 Canal.ipt:114 ↔ 0008-10-2011 DIN 7984 - M5 x 16.ipt:115
- [Insert]: 0008-10-2011 DIN 7984 - M5 x 16.ipt:115 ↔ 0008-10-2012 DIN 125 - A 5.3.ipt:116
- Insert:94: 0008-10-030 Suport L.ipt:23 ↔ 0008-10-2012 DIN 125 - A 5.3.ipt:83
- Insert:95: 0008-10-030 Suport L.ipt:23 ↔ 0008-10-2012 DIN 125 - A 5.3.ipt:89
- Insert:96: 0008-10-031 Suport L + placa.ipt:22 ↔ 0008-10-2012 DIN 125 - A 5.3.ipt:86
- Insert:97: 0008-10-031 Suport L + placa.ipt:22 ↔ 0008-10-2012 DIN 125 - A 5.3.ipt:92
- Insert:98: 0008-10-031 Suport L + placa.ipt:22 ↔ 0008-10-2012 DIN 125 - A 5.3.ipt:95
- Insert:99: 0008-10-031 Suport L + placa.ipt:22 ↔ 0008-10-2012 DIN 125 - A 5.3.ipt:116
- Insert:100: 0008-10-031 Suport L + placa.ipt:22 ↔ 0008-10-2012 DIN 125 - A 5.3.ipt:101
- Insert:101: 0008-10-031 Suport L + placa.ipt:22 ↔ 0008-10-2012 DIN 125 - A 5.3.ipt:104
- Insert:102: 0008-10-031 Suport L + placa.ipt:22 ↔ 0008-10-2012 DIN 125 - A 5.3.ipt:98
- Insert:103: 0008-10-031 Suport L + placa.ipt:22 ↔ 0008-10-2012 DIN 125 - A 5.3.ipt:113
- Insert:104: 0008-10-030 Suport L.ipt:24 ↔ 0008-10-2012 DIN 125 - A 5.3.ipt:110
- Insert:105: 0008-10-030 Suport L.ipt:24 ↔ 0008-10-2012 DIN 125 - A 5.3.ipt:107
- [Insert] (-5 mm): 0008-10-2010 M 5 Canal.ipt:117 ↔ 0008-10-2011 DIN 7984 - M5 x 16.ipt:118
- [Insert]: 0008-10-2011 DIN 7984 - M5 x 16.ipt:118 ↔ 0008-10-2012 DIN 125 - A 5.3.ipt:119
- [Insert] (-5 mm): 0008-10-2010 M 5 Canal.ipt:120 ↔ 0008-10-2011 DIN 7984 - M5 x 16.ipt:121
- [Insert]: 0008-10-2011 DIN 7984 - M5 x 16.ipt:121 ↔ 0008-10-2012 DIN 125 - A 5.3.ipt:122
- [Insert] (-5 mm): 0008-10-2010 M 5 Canal.ipt:123 ↔ 0008-10-2011 DIN 7984 - M5 x 16.ipt:124
- [Insert]: 0008-10-2011 DIN 7984 - M5 x 16.ipt:124 ↔ 0008-10-2012 DIN 125 - A 5.3.ipt:125
- [Insert] (-5 mm): 0008-10-2010 M 5 Canal.ipt:126 ↔ 0008-10-2011 DIN 7984 - M5 x 16.ipt:127
- [Insert]: 0008-10-2011 DIN 7984 - M5 x 16.ipt:127 ↔ 0008-10-2012 DIN 125 - A 5.3.ipt:128
- Insert:114: 0008-10-053 picior.ipt:32 ↔ 0008-10-2012 DIN 125 - A 5.3.ipt:119
- Insert:115: 0008-10-053 picior.ipt:29 ↔ 0008-10-2012 DIN 125 - A 5.3.ipt:122
- Insert:116: 0008-10-053 picior.ipt:30 ↔ 0008-10-2012 DIN 125 - A 5.3.ipt:125
- Insert:117: 0008-10-053 picior.ipt:31 ↔ 0008-10-2012 DIN 125 - A 5.3.ipt:128
- [Insert] (-5 mm): 0008-10-2010 M 5 Canal.ipt:129 ↔ 0008-10-2011 DIN 7984 - M5 x 16.ipt:130
- [Insert]: 0008-10-2011 DIN 7984 - M5 x 16.ipt:130 ↔ 0008-10-2012 DIN 125 - A 5.3.ipt:131
- [Insert] (-5 mm): 0008-10-2010 M 5 Canal.ipt:132 ↔ 0008-10-2011 DIN 7984 - M5 x 16.ipt:133
- [Insert]: 0008-10-2011 DIN 7984 - M5 x 16.ipt:133 ↔ 0008-10-2012 DIN 125 - A 5.3.ipt:134
- [Insert] (-5 mm): 0008-10-2010 M 5 Canal.ipt:135 ↔ 0008-10-2011 DIN 7984 - M5 x 16.ipt:136
- [Insert]: 0008-10-2011 DIN 7984 - M5 x 16.ipt:136 ↔ 0008-10-2012 DIN 125 - A 5.3.ipt:137
- [Insert] (-5 mm): 0008-10-2010 M 5 Canal.ipt:138 ↔ 0008-10-2011 DIN 7984 - M5 x 16.ipt:139
- [Insert]: 0008-10-2011 DIN 7984 - M5 x 16.ipt:139 ↔ 0008-10-2012 DIN 125 - A 5.3.ipt:140
- [Insert] (-5 mm): 0008-10-2010 M 5 Canal.ipt:141 ↔ 0008-10-2011 DIN 7984 - M5 x 16.ipt:142
- [Insert]: 0008-10-2011 DIN 7984 - M5 x 16.ipt:142 ↔ 0008-10-2012 DIN 125 - A 5.3.ipt:143
- [Insert] (-5 mm): 0008-10-2010 M 5 Canal.ipt:144 ↔ 0008-10-2011 DIN 7984 - M5 x 16.ipt:145
- [Insert]: 0008-10-2011 DIN 7984 - M5 x 16.ipt:145 ↔ 0008-10-2012 DIN 125 - A 5.3.ipt:146
- [Insert] (-5 mm): 0008-10-2010 M 5 Canal.ipt:147 ↔ 0008-10-2011 DIN 7984 - M5 x 16.ipt:148
- [Insert]: 0008-10-2011 DIN 7984 - M5 x 16.ipt:148 ↔ 0008-10-2012 DIN 125 - A 5.3.ipt:149
- [Insert] (-5 mm): 0008-10-2010 M 5 Canal.ipt:150 ↔ 0008-10-2011 DIN 7984 - M5 x 16.ipt:151
- [Insert]: 0008-10-2011 DIN 7984 - M5 x 16.ipt:151 ↔ 0008-10-2012 DIN 125 - A 5.3.ipt:152
- [Insert] (-5 mm): 0008-10-2010 M 5 Canal.ipt:153 ↔ 0008-10-2011 DIN 7984 - M5 x 16.ipt:154
- [Insert]: 0008-10-2011 DIN 7984 - M5 x 16.ipt:154 ↔ 0008-10-2012 DIN 125 - A 5.3.ipt:155
- [Insert] (-5 mm): 0008-10-2010 M 5 Canal.ipt:156 ↔ 0008-10-2011 DIN 7984 - M5 x 16.ipt:157
- [Insert]: 0008-10-2011 DIN 7984 - M5 x 16.ipt:157 ↔ 0008-10-2012 DIN 125 - A 5.3.ipt:158
- [Insert] (-5 mm): 0008-10-2010 M 5 Canal.ipt:159 ↔ 0008-10-2011 DIN 7984 - M5 x 16.ipt:160
- [Insert]: 0008-10-2011 DIN 7984 - M5 x 16.ipt:160 ↔ 0008-10-2012 DIN 125 - A 5.3.ipt:161
- [Insert] (-5 mm): 0008-10-2010 M 5 Canal.ipt:162 ↔ 0008-10-2011 DIN 7984 - M5 x 16.ipt:163
- [Insert]: 0008-10-2011 DIN 7984 - M5 x 16.ipt:163 ↔ 0008-10-2012 DIN 125 - A 5.3.ipt:164
- Insert:142: 0008-10-030 Suport L.ipt:20 ↔ 0008-10-2012 DIN 125 - A 5.3.ipt:164
- Insert:143: 0008-10-030 Suport L.ipt:20 ↔ 0008-10-2012 DIN 125 - A 5.3.ipt:137
- Insert:144: 0008-10-031 Suport L + placa.ipt:19 ↔ 0008-10-2012 DIN 125 - A 5.3.ipt:134
- Insert:145: 0008-10-031 Suport L + placa.ipt:19 ↔ 0008-10-2012 DIN 125 - A 5.3.ipt:131
- Insert:146: 0008-10-031 Suport L + placa.ipt:19 ↔ 0008-10-2012 DIN 125 - A 5.3.ipt:140
- Insert:147: 0008-10-031 Suport L + placa.ipt:19 ↔ 0008-10-2012 DIN 125 - A 5.3.ipt:146
- Insert:148: 0008-10-031 Suport L + placa.ipt:19 ↔ 0008-10-2012 DIN 125 - A 5.3.ipt:161
- Insert:149: 0008-10-031 Suport L + placa.ipt:19 ↔ 0008-10-2012 DIN 125 - A 5.3.ipt:158
- Insert:150: 0008-10-031 Suport L + placa.ipt:19 ↔ 0008-10-2012 DIN 125 - A 5.3.ipt:143
- Insert:151: 0008-10-030 Suport L.ipt:21 ↔ 0008-10-2012 DIN 125 - A 5.3.ipt:155
- Insert:152: 0008-10-030 Suport L.ipt:21 ↔ 0008-10-2012 DIN 125 - A 5.3.ipt:152
- Insert:153: 0008-10-031 Suport L + placa.ipt:19 ↔ 0008-10-2012 DIN 125 - A 5.3.ipt:149
- [Insert] (-5 mm): 0008-10-2010 M 5 Canal.ipt:165 ↔ 0008-10-2011 DIN 7984 - M5 x 16.ipt:166
- [Insert]: 0008-10-2011 DIN 7984 - M5 x 16.ipt:166 ↔ 0008-10-2012 DIN 125 - A 5.3.ipt:167
- [Insert] (-5 mm): 0008-10-2010 M 5 Canal.ipt:168 ↔ 0008-10-2011 DIN 7984 - M5 x 16.ipt:169
- [Insert]: 0008-10-2011 DIN 7984 - M5 x 16.ipt:169 ↔ 0008-10-2012 DIN 125 - A 5.3.ipt:170
- [Insert] (-5 mm): 0008-10-2010 M 5 Canal.ipt:171 ↔ 0008-10-2011 DIN 7984 - M5 x 16.ipt:172
- [Insert]: 0008-10-2011 DIN 7984 - M5 x 16.ipt:172 ↔ 0008-10-2012 DIN 125 - A 5.3.ipt:173
- [Insert] (-5 mm): 0008-10-2010 M 5 Canal.ipt:174 ↔ 0008-10-2011 DIN 7984 - M5 x 16.ipt:175
- [Insert]: 0008-10-2011 DIN 7984 - M5 x 16.ipt:175 ↔ 0008-10-2012 DIN 125 - A 5.3.ipt:176
- Insert:162: 0008-10-032 Suport cadru si axa Z.ipt:28 ↔ 0008-10-2012 DIN 125 - A 5.3.ipt:167
- Insert:163: 0008-10-032 Suport cadru si axa Z.ipt:28 ↔ 0008-10-2012 DIN 125 - A 5.3.ipt:170
- Insert:164: 0008-10-032 Suport cadru si axa Z.ipt:28 ↔ 0008-10-2012 DIN 125 - A 5.3.ipt:176
- Insert:165: 0008-10-032 Suport cadru si axa Z.ipt:28 ↔ 0008-10-2012 DIN 125 - A 5.3.ipt:173
- [Insert] (-5 mm): 0008-10-2010 M 5 Canal.ipt:177 ↔ 0008-10-2011 DIN 7984 - M5 x 16.ipt:178
- [Insert]: 0008-10-2011 DIN 7984 - M5 x 16.ipt:178 ↔ 0008-10-2012 DIN 125 - A 5.3.ipt:179
- [Insert] (-5 mm): 0008-10-2010 M 5 Canal.ipt:180 ↔ 0008-10-2011 DIN 7984 - M5 x 16.ipt:181
- [Insert]: 0008-10-2011 DIN 7984 - M5 x 16.ipt:181 ↔ 0008-10-2012 DIN 125 - A 5.3.ipt:182
- [Insert] (-5 mm): 0008-10-2010 M 5 Canal.ipt:183 ↔ 0008-10-2011 DIN 7984 - M5 x 16.ipt:184
- [Insert]: 0008-10-2011 DIN 7984 - M5 x 16.ipt:184 ↔ 0008-10-2012 DIN 125 - A 5.3.ipt:185
- [Insert] (-5 mm): 0008-10-2010 M 5 Canal.ipt:186 ↔ 0008-10-2011 DIN 7984 - M5 x 16.ipt:187
- [Insert]: 0008-10-2011 DIN 7984 - M5 x 16.ipt:187 ↔ 0008-10-2012 DIN 125 - A 5.3.ipt:188
- Insert:174: 0008-10-032 Suport cadru si axa Z.ipt:25 ↔ 0008-10-2012 DIN 125 - A 5.3.ipt:179
- Insert:175: 0008-10-032 Suport cadru si axa Z.ipt:25 ↔ 0008-10-2012 DIN 125 - A 5.3.ipt:185
- Insert:176: 0008-10-032 Suport cadru si axa Z.ipt:25 ↔ 0008-10-2012 DIN 125 - A 5.3.ipt:182
- Insert:177: 0008-10-032 Suport cadru si axa Z.ipt:25 ↔ 0008-10-2012 DIN 125 - A 5.3.ipt:188
- Insert:178 (-5 mm): 0008-10-2010 M 5 Canal.ipt:189 ↔ 0008-10-2013 DIN 7984 - M5 x 20.ipt:191